# Autodesk Inventor assembly: Motor Assembly
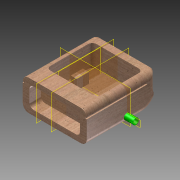
[picture p0: Inventor's stored thumbnail of the model, 180x180]
Saved by Autodesk Inventor 2015 (Build 190159000, 159)
## iProperties
Created: 2018-02-26
Part Number: Motor Assembly
Document SubType Name: Assembly
Designer: Administrator
Author: Administrator
## Documents named in this file (3)
- L:\IED 9th\Automoblox\7.4 Exact Parts\Motor Assembly.iam
- L:\IED 9th\Automoblox\7.4 Exact Parts\Motor Bed.ipt
- L:\IED 9th\Automoblox\7.4 Exact Parts\Motor Axle.ipt
## Components (2 placed, 2 different names)
1. Motor Bed:1 — Mate:1, Mate:2, Flush:1
2. Motor Axle:1 — Mate:1, Mate:2, Flush:2
## Relationships (4: Mate 2, Flush 2)
- Mate:1: Motor Bed:1 ↔ Motor Axle:1
- Mate:2: Motor Bed:1 ↔ Motor Axle:1
- Flush:1 (12.7 mm): Motor Bed:1
- Flush:2 (-32.385 mm): Motor Axle:1
